# Autodesk Inventor assembly: Khung máy
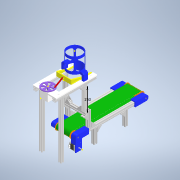
[picture p0: Inventor's stored thumbnail of the model, 180x180]
Saved by Autodesk Inventor 2020 (Build 240168000, 168)
## iProperties
Created: 2022-12-09
Part Number: Khung máy
Document SubType Name: Assembly
Designer: ADMIN
_SolveAssemblyDoc: Frame Generator Solve Assembly
_Version: 15.0.0
Author: ADMIN
## Documents named in this file (6)
- D:\Do-an-tot-nghiep\Inventor\Khung máy.iam
- D:\Do-an-tot-nghiep\Inventor\Băng chuyền.iam
- D:\Do-an-tot-nghiep\Inventor\Cơ cấu gạt cốc.iam
- D:\Do-an-tot-nghiep\Inventor\Thanh đỡ.ipt
- D:\Do-an-tot-nghiep\Inventor\Khung máy\Frame\Frame 1670596914194.iam
- D:\Do-an-tot-nghiep\Inventor\KeGoc2020_SuaLai.ipt
## Components (20 placed, 5 different names)
1. Cơ cấu gạt cốc:1 [sub-assembly] — Flush:2, Flush:4, Flush:6, Mate:2, Mate:7, Mate:10, Flush:11, Flush:12, Mate:26, Flush:18, Mate:27, Mate:28, Mate:29, Flush:19
2. Băng chuyền:2 [sub-assembly] — Flush:1, Mate:1, Mate:3, Mate:4, Mate:5, Mate:6, Mate:12, Mate:13, Mate:14, Mate:15, Flush:7, Flush:8, Flush:9, Flush:10, Mate:16, Mate:17, Flush:13, Mate:18, Mate:19, Flush:14, Mate:20, Mate:21, Mate:22, Flush:16, Mate:24, Mate:25, Flush:17, Flush:20, Mate:30, Mate:31, Mate:32, Flush:21
3. Thanh đỡ:1
4. Frame 1670596914194:1 [sub-assembly] — Flush:5, Flush:6, Mate:8, Mate:9, Flush:16, Mate:32
5. Frame 1670596914194:2 [sub-assembly] — Flush:4, Flush:5, Mate:1, Mate:2, Mate:11, Flush:15, Mate:23
6. KeGoc2020_SuaLai:1 — Mate:12, Mate:13, Flush:8
7. KeGoc2020_SuaLai:2 — Mate:14, Mate:15, Flush:7
8. KeGoc2020_SuaLai:3 — Mate:9, Flush:9, Mate:17
9. KeGoc2020_SuaLai:4 — Flush:15, Mate:22, Mate:23
10. KeGoc2020_SuaLai:5 — Flush:10, Mate:16
11. KeGoc2020_SuaLai:6 — Mate:5, Mate:6
12. KeGoc2020_SuaLai:7 — Mate:3, Mate:4, Flush:21
13. KeGoc2020_SuaLai:8 — Flush:14, Mate:20, Mate:21
14. KeGoc2020_SuaLai:9 — Mate:7, Mate:8, Flush:11
15. KeGoc2020_SuaLai:10 — Flush:13, Mate:18, Mate:19
16. KeGoc2020_SuaLai:11 — Mate:10, Mate:11, Flush:12
17. KeGoc2020_SuaLai:12 — Mate:24, Mate:25, Flush:17
18. KeGoc2020_SuaLai:16 — Mate:28, Mate:29, Flush:19
19. KeGoc2020_SuaLai:17 — Flush:20, Mate:30, Mate:31
20. KeGoc2020_SuaLai:18 — Mate:26, Flush:18, Mate:27
## Relationships (53: Mate 32, Flush 21)
- Flush:1 (-48 mm): Băng chuyền:2
- Flush:2 (-76 mm): Cơ cấu gạt cốc:1
- Flush:3
- Flush:4: Cơ cấu gạt cốc:1 ↔ Frame 1670596914194:2
- Flush:5: Frame 1670596914194:1 ↔ Frame 1670596914194:2
- Mate:1: Băng chuyền:2 ↔ Frame 1670596914194:2
- Flush:6: Cơ cấu gạt cốc:1 ↔ Frame 1670596914194:1
- Mate:2: Cơ cấu gạt cốc:1 ↔ Frame 1670596914194:2
- Mate:3: Băng chuyền:2 ↔ KeGoc2020_SuaLai:7
- Mate:4: Băng chuyền:2 ↔ KeGoc2020_SuaLai:7
- Mate:5: Băng chuyền:2 ↔ KeGoc2020_SuaLai:6
- Mate:6: Băng chuyền:2 ↔ KeGoc2020_SuaLai:6
- Mate:7: Cơ cấu gạt cốc:1 ↔ KeGoc2020_SuaLai:9
- Mate:8: Frame 1670596914194:1 ↔ KeGoc2020_SuaLai:9
- Mate:9: Frame 1670596914194:1 ↔ KeGoc2020_SuaLai:3
- Mate:10: Cơ cấu gạt cốc:1 ↔ KeGoc2020_SuaLai:11
- Mate:11: Frame 1670596914194:2 ↔ KeGoc2020_SuaLai:11
- Mate:12: Băng chuyền:2 ↔ KeGoc2020_SuaLai:1
- Mate:13: Băng chuyền:2 ↔ KeGoc2020_SuaLai:1
- Mate:14: Băng chuyền:2 ↔ KeGoc2020_SuaLai:2
- Mate:15: Băng chuyền:2 ↔ KeGoc2020_SuaLai:2
- Flush:7: Băng chuyền:2 ↔ KeGoc2020_SuaLai:2
- Flush:8: Băng chuyền:2 ↔ KeGoc2020_SuaLai:1
- Flush:9: Băng chuyền:2 ↔ KeGoc2020_SuaLai:3
- Flush:10: Băng chuyền:2 ↔ KeGoc2020_SuaLai:5
- Mate:16: Băng chuyền:2 ↔ KeGoc2020_SuaLai:5
- Flush:11: Cơ cấu gạt cốc:1 ↔ KeGoc2020_SuaLai:9
- Flush:12: Cơ cấu gạt cốc:1 ↔ KeGoc2020_SuaLai:11
- Mate:17: Băng chuyền:2 ↔ KeGoc2020_SuaLai:3
- Flush:13: Băng chuyền:2 ↔ KeGoc2020_SuaLai:10
- Mate:18: Băng chuyền:2 ↔ KeGoc2020_SuaLai:10
- Mate:19: Băng chuyền:2 ↔ KeGoc2020_SuaLai:10
- Flush:14: Băng chuyền:2 ↔ KeGoc2020_SuaLai:8
- Mate:20: Băng chuyền:2 ↔ KeGoc2020_SuaLai:8
- Mate:21: Băng chuyền:2 ↔ KeGoc2020_SuaLai:8
- Flush:15: Frame 1670596914194:2 ↔ KeGoc2020_SuaLai:4
- Mate:22: Băng chuyền:2 ↔ KeGoc2020_SuaLai:4
- Mate:23: Frame 1670596914194:2 ↔ KeGoc2020_SuaLai:4
- Flush:16: Băng chuyền:2 ↔ Frame 1670596914194:1
- Mate:24: Băng chuyền:2 ↔ KeGoc2020_SuaLai:12
- Mate:25: Băng chuyền:2 ↔ KeGoc2020_SuaLai:12
- Flush:17: Băng chuyền:2 ↔ KeGoc2020_SuaLai:12
- Mate:26: Cơ cấu gạt cốc:1 ↔ KeGoc2020_SuaLai:18
- Flush:18: Cơ cấu gạt cốc:1 ↔ KeGoc2020_SuaLai:18
- Mate:27: Cơ cấu gạt cốc:1 ↔ KeGoc2020_SuaLai:18
- Mate:28: Cơ cấu gạt cốc:1 ↔ KeGoc2020_SuaLai:16
- Mate:29: Cơ cấu gạt cốc:1 ↔ KeGoc2020_SuaLai:16
- Flush:19: Cơ cấu gạt cốc:1 ↔ KeGoc2020_SuaLai:16
- Flush:20: Băng chuyền:2 ↔ KeGoc2020_SuaLai:17
- Mate:30: Băng chuyền:2 ↔ KeGoc2020_SuaLai:17
- Mate:31: Băng chuyền:2 ↔ KeGoc2020_SuaLai:17
- Mate:32: Băng chuyền:2 ↔ Frame 1670596914194:1
- Flush:21: Băng chuyền:2 ↔ KeGoc2020_SuaLai:7
